# Autodesk Inventor assembly: ThArLampCase
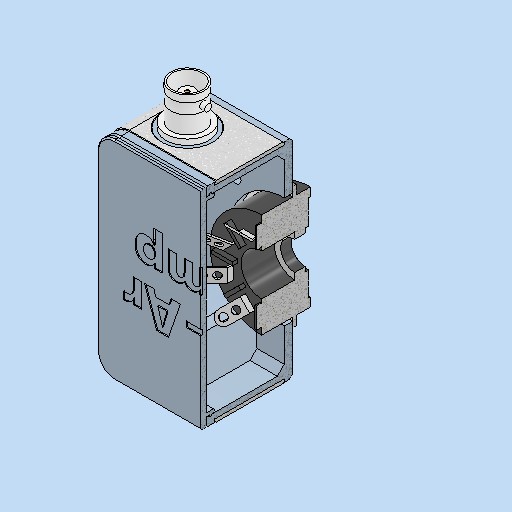
[picture p0: Inventor's stored thumbnail of the model, 512x512]
Saved by Autodesk Inventor 2025 (Build 290162000, 162)
## iProperties
Created: 2025-03-14
Part Number: ThArLampCase
Document SubType Name: Assembly
Designer: kuzmin
Author: kuzmin
## Documents named in this file (6)
- C:\Users\queez\Dropbox\Drawings\PIHTI\ElectricAdapters\ThArLamp\ThArLampCase.iam
- C:\Users\queez\Dropbox\Drawings\PIHTI\ElectricAdapters\ThArLamp\LampConnectorEnclosure.ipt
- C:\Users\queez\Dropbox\Drawings\PIHTI\ElectricAdapters\ThArLamp\LampConnectorEnclosure-lid.ipt
- C:\Users\queez\Dropbox\Drawings\PIHTI\ContentCenter\Electrics\PL08.ipt
- C:\Users\queez\Dropbox\Drawings\PIHTI\ContentCenter\Electrics\BNC Connector.ipt
- C:\Users\queez\Dropbox\Drawings\PIHTI\ElectricAdapters\ThArLamp\15kOhmResistor.ipt
## Components (6 placed, 5 different names)
1. LampConnectorEnclosure:1 — Rigid:1, Mate:1, Mate:2, Rotational:1, Flush:1, Flush:2
2. LampConnectorEnclosure-lid:1 — Rigid:1
3. PL08:1 — Mate:1, Mate:2
4. BNC Connector:1 — Rotational:1
5. 15kOhmResistor:1
6. 15kOhmResistor:2
## Relationships (6: Mate 2, Flush 2, WeldJoint 1, RevoluteJoint 1)
- Rigid:1 [WeldJoint]: LampConnectorEnclosure:1 ↔ LampConnectorEnclosure-lid:1
- Mate:1: LampConnectorEnclosure:1 ↔ PL08:1
- Mate:2: LampConnectorEnclosure:1 ↔ PL08:1
- Rotational:1 [RevoluteJoint]: LampConnectorEnclosure:1 ↔ BNC Connector:1
- Flush:1: LampConnectorEnclosure:1
- Flush:2: LampConnectorEnclosure:1
